# Autodesk Inventor assembly: Tool Dock Assembly
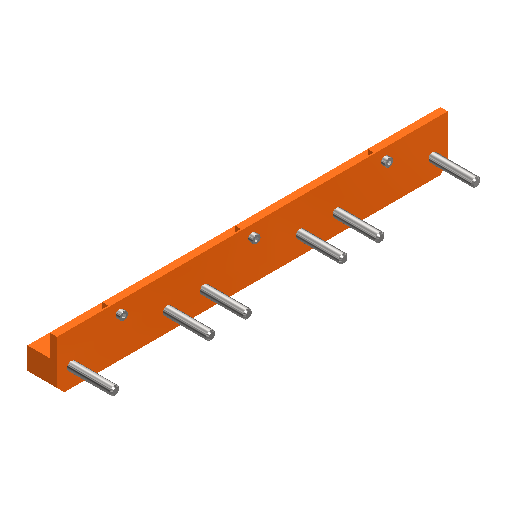
[picture p0: Inventor's stored thumbnail of the model, 512x512]
Saved by Autodesk Inventor 2023.2 (Build 272271000, 271)
## iProperties
Created: 2023-02-06
Part Number: Tool Dock Assembly
Document SubType Name: Assembly
Designer: remop
Author: remop
## Documents named in this file (5)
- C:\Users\remop\OneDrive\Documents\Inventor\3D Printers\LuEVO\Mk5_FullKinematic\Tool Dock Assembly.iam
- C:\Users\remop\OneDrive\Documents\Inventor\3D Printers\LuEVO\Mk5_FullKinematic\Tool Dock Base.ipt
- C:\Users\remop\OneDrive\Documents\Inventor\Content Center Files\R2023\en-US\AS 1420\AS 1420 - 1973 - M3 x 8.ipt
- C:\Users\remop\OneDrive\Documents\Inventor\3D Printers\LuEVO\Mk5_FullKinematic\Tool Dock Bolt.ipt
- C:\Users\remop\OneDrive\Documents\Inventor\Content Center Files\R2023\en-US\AS 1420\AS 1420 - 1973 - M3 x 12.ipt
## Components (13 placed, 4 different names)
1. Tool Dock Base:1 — Insert:1, Insert:2, Insert:3, Rigid:8, Rigid:9, Rigid:10, Rigid:11, Rigid:12, Rigid:13, Rigid:14, Rigid:15, Rigid:16
2. AS 1420 - Metric M3 x 8:1 — Insert:1
3. AS 1420 - Metric M3 x 8:2 — Insert:2
4. AS 1420 - Metric M3 x 8:3 — Insert:3
5. Tool Dock Bolt:1 — Rigid:12
6. Tool Dock Bolt:2 — Rigid:14
7. Tool Dock Bolt:3 — Rigid:16
8. Tool Dock Bolt:4 — Rigid:15
9. Tool Dock Bolt:5 — Rigid:11
10. Tool Dock Bolt:6 — Rigid:13
11. AS 1420 - Metric M3 x 12:1 — Rigid:8
12. AS 1420 - Metric M3 x 12:2 — Rigid:10
13. AS 1420 - Metric M3 x 12:3 — Rigid:9
## Relationships (12: WeldJoint 9, Insert 3)
- Insert:1: Tool Dock Base:1 ↔ AS 1420 - Metric M3 x 8:1
- Insert:2: Tool Dock Base:1 ↔ AS 1420 - Metric M3 x 8:2
- Insert:3: Tool Dock Base:1 ↔ AS 1420 - Metric M3 x 8:3
- Rigid:8 [WeldJoint] (2 mm): Tool Dock Base:1 ↔ AS 1420 - Metric M3 x 12:1
- Rigid:9 [WeldJoint] (2 mm): Tool Dock Base:1 ↔ AS 1420 - Metric M3 x 12:3
- Rigid:10 [WeldJoint] (2 mm): Tool Dock Base:1 ↔ AS 1420 - Metric M3 x 12:2
- Rigid:11 [WeldJoint] (10 mm): Tool Dock Base:1 ↔ Tool Dock Bolt:5
- Rigid:12 [WeldJoint] (10 mm): Tool Dock Base:1 ↔ Tool Dock Bolt:1
- Rigid:13 [WeldJoint] (10 mm): Tool Dock Base:1 ↔ Tool Dock Bolt:6
- Rigid:14 [WeldJoint] (10 mm): Tool Dock Base:1 ↔ Tool Dock Bolt:2
- Rigid:15 [WeldJoint] (-10 mm): Tool Dock Base:1 ↔ Tool Dock Bolt:4
- Rigid:16 [WeldJoint] (10 mm): Tool Dock Base:1 ↔ Tool Dock Bolt:3
